# Autodesk Inventor assembly: Transmission par courroie trapézoïdale
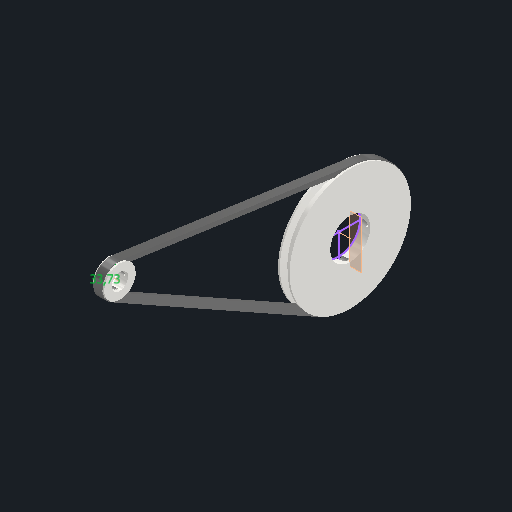
[picture p0: Inventor's stored thumbnail of the model, 512x512]
Saved by Autodesk Inventor 2026.2 (Build 302298010, 298A)
## iProperties
ClientObjectVersion: 1
Created: 2026-03-31
Part Number: Transmission par courroie trapézoïdale
Document SubType Name: Assembly
Designer: romai
Author: romai
## Documents named in this file (4)
- D:\Downloads\LogicielMaster\Inventor\Enssemble\BancEcoShell\BancEcoShell\Design Accelerator\Transmission par courroie trapézoïdale2.iam
- D:\Downloads\LogicielMaster\Inventor\Enssemble\BancEcoShell\BancEcoShell\Design Accelerator\Courroie trapézoïdale2.ipt
- D:\Downloads\LogicielMaster\Inventor\Enssemble\BancEcoShell\BancEcoShell\Design Accelerator\Poulie à gorge12.ipt
- D:\Downloads\LogicielMaster\Inventor\Enssemble\BancEcoShell\BancEcoShell\Design Accelerator\Poulie à gorge22.ipt
## Components (3 placed, 3 different names)
1. Poulie à gorge1:1 — Affleurement:1, Placage:1, Rotation:1
2. Poulie à gorge2:1 — Affleurement:2, Placage:2, Rotation:1
3. Courroie trapézoïdale:1 — Affleurement:1, Placage:1, Affleurement:2, Placage:2
## Component patterns: (1 elements, first: Courroie trapézoïdale:1)
## Relationships (5: Flush 2, Mate 2, RelateRotation 1)
- Affleurement:1 [Flush]: Poulie à gorge1:1 ↔ Courroie trapézoïdale:1
- Placage:1 [Mate]: Poulie à gorge1:1 ↔ Courroie trapézoïdale:1
- Affleurement:2 [Flush]: Poulie à gorge2:1 ↔ Courroie trapézoïdale:1
- Placage:2 [Mate]: Poulie à gorge2:1 ↔ Courroie trapézoïdale:1
- Rotation:1 [RelateRotation] (0.2502 ul): Poulie à gorge1:1 ↔ Poulie à gorge2:1
